# Autodesk Inventor assembly: цепь
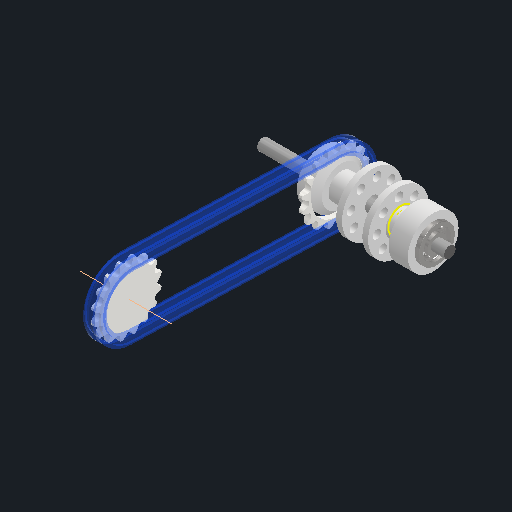
[picture p0: Inventor's stored thumbnail of the model, 512x512]
Saved by Autodesk Inventor 2025 (Build 290162000, 162)
## iProperties
Created: 2024-07-09
Part Number: цепь
Document SubType Name: Assembly
Designer: Phantom
Author: Phantom
## Documents named in this file (6)
- C:\Users\GameHD\Desktop\что-то нужное\Phantom16950\цепь.iam
- C:\Users\GameHD\Desktop\что-то нужное\Phantom16950\Цепной привод2.iam
- C:\Users\GameHD\Desktop\что-то нужное\Phantom16950\втулка для подш 2 часть.ipt
- C:\Users\GameHD\Desktop\что-то нужное\Phantom16950\втулка для подш.ipt
- C:\Users\GameHD\Desktop\что-то нужное\Phantom16950\Деталь_64.ipt
- C:\Users\GameHD\Desktop\что-то нужное\Phantom16950\BS 290 SKF - SKF 626-RZ.ipt
## Components (6 placed, 5 different names)
1. Цепной привод:1 [sub-assembly]
2. втулка для подш 2 часть:1 — Заподлицо:2, Совмещение:11, Совмещение:12, Совмещение:15
3. втулка для подш:1 — Совмещение:12
4. Деталь_64:1 — Совмещение:10, Заподлицо:2, Совмещение:11, Совмещение:14
5. BS 290 SKF - SKF 626-RZ:1 — Совмещение:14, Совмещение:15
6. BS 290 SKF - SKF 626-RZ:2 — Совмещение:10
## Relationships (6: Mate 5, Flush 1)
- Совмещение:10 [Mate]: Деталь_64:1 ↔ BS 290 SKF - SKF 626-RZ:2
- Заподлицо:2 [Flush] (10.245 mm): втулка для подш 2 часть:1 ↔ Деталь_64:1
- Совмещение:11 [Mate]: втулка для подш 2 часть:1 ↔ Деталь_64:1
- Совмещение:12 [Mate]: втулка для подш 2 часть:1 ↔ втулка для подш:1
- Совмещение:14 [Mate]: Деталь_64:1 ↔ BS 290 SKF - SKF 626-RZ:1
- Совмещение:15 [Mate]: втулка для подш 2 часть:1 ↔ BS 290 SKF - SKF 626-RZ:1
